# Autodesk Inventor assembly: assemEdit
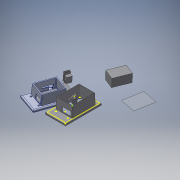
[picture p0: Inventor's stored thumbnail of the model, 180x180]
Saved by Autodesk Inventor 2019 (Build 230136000, 136)
## iProperties
Created: 2019-06-25
Part Number: assemEdit
Document SubType Name: Assembly
Designer: Daniel
Author: Daniel
## Documents named in this file (9)
- C:\Users\Shman\Desktop\Radwatch\newtouchscreen\assemEdit.iam
- C:\Users\Shman\Desktop\Radwatch\newtouchscreen\aqisensor.ipt
- C:\Users\Shman\Desktop\Radwatch\newtouchscreen\co2sensor.ipt
- C:\Users\Shman\Desktop\Radwatch\newtouchscreen\rpibox.ipt
- C:\Users\Shman\Desktop\Radwatch\newtouchscreen\screen.ipt
- C:\Users\Shman\Desktop\Radwatch\newtouchscreen\touchscreenCase.ipt
- C:\Users\Shman\Desktop\Radwatch\Portable Design\touchscreen cover.ipt
- C:\Users\Shman\Desktop\Radwatch\newtouchscreen\battery.ipt
- C:\Users\Shman\Desktop\Radwatch\newtouchscreen\acrylic cover.ipt
## Components (8 placed, 8 different names)
1. aqisensor:1 — Mate:5, Mate:6, Tangent:2, Angle:1
2. co2sensor:1 — Mate:6, Angle:1
3. rpibox:1 — Mate:3
4. screen:1 — Mate:2, Mate:3, Flush:1, Flush:2
5. touchscreenCase:1
6. touchscreen cover:1 — Mate:1, Mate:2, Flush:1, Flush:2, Mate:4, Tangent:1, Mate:5, Tangent:2, Mate:7
7. battery:1 — Mate:1, Mate:4, Tangent:1
8. acrylic cover:1 — Mate:7
## Relationships (12: Mate 7, Flush 2, Tangent 2, Angle 1)
- Mate:1: touchscreen cover:1 ↔ battery:1
- Mate:2: screen:1 ↔ touchscreen cover:1
- Mate:3: rpibox:1 ↔ screen:1
- Flush:1 (0.508 mm): screen:1 ↔ touchscreen cover:1
- Flush:2 (0.762 mm): screen:1 ↔ touchscreen cover:1
- Mate:4: touchscreen cover:1 ↔ battery:1
- Tangent:1: touchscreen cover:1 ↔ battery:1
- Mate:5: aqisensor:1 ↔ touchscreen cover:1
- Mate:6: aqisensor:1 ↔ co2sensor:1
- Tangent:2: aqisensor:1 ↔ touchscreen cover:1
- Angle:1 (0 deg): aqisensor:1 ↔ co2sensor:1
- Mate:7: touchscreen cover:1 ↔ acrylic cover:1
